# Autodesk Inventor assembly: Working Simlation and Assembly
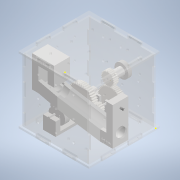
[picture p0: Inventor's stored thumbnail of the model, 180x180]
Saved by Autodesk Inventor 2021 (Build 250183000, 183)
## iProperties
Created: 2021-04-14
Part Number: Working Simlation and Assembly
Document SubType Name: Assembly
Designer: Nabeel Azafer
Author: Nabeel Azafer
## Documents named in this file (24)
- C:\Uni\Sem1\334\Project A\New Founding\ZIP\Working Simlation and Assembly.iam
- C:\Uni\Sem1\334\Project A\Spur Gear Large 4-1.ipt
- C:\Uni\Sem1\334\Project A\Spur Gear Small 4-1.ipt
- C:\Uni\Sem1\334\Project A\Block.ipt
- C:\Uni\Sem1\334\Project A\Cam.ipt
- C:\Uni\Sem1\334\Project A\Extra Shaft.ipt
- C:\Uni\Sem1\334\Project A\Shaft 2.ipt
- C:\Uni\Sem1\334\Project A\Spur Gear Small 2-1.ipt
- C:\Uni\Sem1\334\Project A\Spur Gear Large 2-1.ipt
- C:\Uni\Sem1\334\Project A\Input Connection.ipt
- C:\Uni\Sem1\334\Project A\Driveshaft coupling end.ipt
- C:\Uni\Sem1\334\Project A\Box base.ipt
- C:\Uni\Sem1\334\Project A\Box side 2.ipt
- C:\Uni\Sem1\334\Project A\Box side 4.ipt
- C:\Uni\Sem1\334\Project A\Box top.ipt
- C:\Uni\Sem1\334\Project A\Box side 1.ipt
- C:\Uni\Sem1\334\Project A\entry_ramp.ipt
- C:\Uni\Sem1\334\Project A\bottom_part.ipt
- C:\Uni\Sem1\334\Project A\Box_side_3.ipt
- C:\Uni\Sem1\334\Project A\Ball.ipt
- C:\Uni\Sem1\334\Project A\Support_1A.ipt
- C:\Uni\Sem1\334\Project A\Support_1B.ipt
- C:\Uni\Sem1\334\Project A\Support_2A.ipt
- C:\Uni\Sem1\334\Project A\Support_2B.ipt
## Components (23 placed, 21 different names)
1. Spur Gear1:1 — Mate:1, Flush:1, Rigid:1, Flush:4, Mate:2, Tangent:1, Rotation:1
2. Block:2 — Flush:2, Flush:3, Mate:24, Mate:25, Transitional:1
3. Cam:1 — Rigid:2, Flush:2, Transitional:1
4. Shaft 2:1 — Rigid:1, Rigid:2
5. Spur Gear2:1 — Flush:4, Mate:2, Tangent:1, Mate:3, Rotation:1, Rigid:3
6. Extra Shaft:2 — Rigid:3, Rigid:4
7. Spur Gear2:2 — Flush:7, Mate:4, Mate:5, Rigid:6, Rotation:2, Rigid:7, Mate:29
8. Spur Gear1:2 — Rigid:4, Flush:7, Mate:4, Rotation:2
9. Input Connection:1 — Rigid:5, Rigid:6, Rigid:7, Mate:28
10. Driveshaft coupling end:1 — Rigid:5
11. Box base:1 — Mate:9, Mate:10, Mate:11, Mate:13, Mate:14, Mate:27, Mate:28, Mate:31, Mate:32, Rigid:10, Rigid:12, Rigid:13
12. Box side 2:1 — Mate:12, Mate:13, Mate:14, Mate:15, Mate:23, Mate:30, Mate:33, Rigid:9
13. Box top:1 — Mate:22, Mate:23, Mate:30
14. Box side 1:1 — Mate:6, Mate:7, Mate:8, Mate:9, Mate:10, Mate:11, Mate:12, Mate:15, Rigid:11
15. Box side 4:2 — Mate:6, Mate:7, Mate:8, Mate:22, Rigid:8, Flush:10, Mate:29
16. entry_ramp:1 — Rigid:8, Mate:24, Mate:25
17. bottom_part:1 — Rigid:9
18. Box_side_3:1 — Mate:31, Mate:32, Mate:33
19. Ball:1
20. Support_1A:1 — Rigid:11
21. Support_1B:1 — Rigid:10, Flush:11
22. Support_2B:1 — Rigid:12
23. Support_2A:2 — Rigid:13
## Relationships (51: Mate 26, WeldJoint 13, Flush 8, RelateRotation 2, Tangent 1, Transitional 1)
- Mate:1: Spur Gear1:1
- Flush:1: Spur Gear1:1
- Rigid:1 [WeldJoint] (16 mm): Spur Gear1:1 ↔ Shaft 2:1
- Rigid:2 [WeldJoint] (-9.5 mm): Cam:1 ↔ Shaft 2:1
- Flush:2 (-4.5 mm): Block:2 ↔ Cam:1
- Flush:3 (-2.5 mm): Block:2
- Flush:4: Spur Gear1:1 ↔ Spur Gear2:1
- Mate:2: Spur Gear1:1 ↔ Spur Gear2:1
- Tangent:1: Spur Gear1:1 ↔ Spur Gear2:1
- Mate:3: Spur Gear2:1
- Rotation:1 [RelateRotation] (0.5 ul): Spur Gear1:1 ↔ Spur Gear2:1
- Rigid:3 [WeldJoint] (6.5 mm): Spur Gear2:1 ↔ Extra Shaft:2
- Rigid:4 [WeldJoint] (-6 mm): Extra Shaft:2 ↔ Spur Gear1:2
- Flush:6 (24.981 mm)
- Flush:7: Spur Gear2:2 ↔ Spur Gear1:2
- Mate:4: Spur Gear2:2 ↔ Spur Gear1:2
- Mate:5: Spur Gear2:2
- Rigid:5 [WeldJoint]: Input Connection:1 ↔ Driveshaft coupling end:1
- Rigid:6 [WeldJoint]: Spur Gear2:2 ↔ Input Connection:1
- Rotation:2 [RelateRotation] (0.5 ul): Spur Gear2:2 ↔ Spur Gear1:2
- Rigid:7 [WeldJoint]: Spur Gear2:2 ↔ Input Connection:1
- Mate:6: Box side 1:1 ↔ Box side 4:2
- Mate:7: Box side 1:1 ↔ Box side 4:2
- Mate:8: Box side 1:1 ↔ Box side 4:2
- Mate:9: Box base:1 ↔ Box side 1:1
- Mate:10: Box base:1 ↔ Box side 1:1
- Mate:11: Box base:1 ↔ Box side 1:1
- Mate:12: Box side 2:1 ↔ Box side 1:1
- Mate:13: Box base:1 ↔ Box side 2:1
- Mate:14: Box base:1 ↔ Box side 2:1
- Mate:15: Box side 2:1 ↔ Box side 1:1
- Mate:22: Box top:1 ↔ Box side 4:2
- Mate:23: Box side 2:1 ↔ Box top:1
- Rigid:8 [WeldJoint]: Box side 4:2 ↔ entry_ramp:1
- Mate:24 (0.5 mm): Block:2 ↔ entry_ramp:1
- Mate:25 (0.5 mm): Block:2 ↔ entry_ramp:1
- Flush:10 (48.343 mm): Box side 4:2
- Mate:27 (24 mm): Box base:1
- Mate:28 (48.516 mm): Input Connection:1 ↔ Box base:1
- Mate:29 (48.343 mm): Spur Gear2:2 ↔ Box side 4:2
- Mate:30: Box side 2:1 ↔ Box top:1
- Mate:31: Box base:1 ↔ Box_side_3:1
- Mate:32: Box base:1 ↔ Box_side_3:1
- Mate:33: Box side 2:1 ↔ Box_side_3:1
- Rigid:9 [WeldJoint]: Box side 2:1 ↔ bottom_part:1
- Rigid:10 [WeldJoint]: Box base:1 ↔ Support_1B:1
- Flush:11 (-2.962 mm): Support_1B:1
- Rigid:11 [WeldJoint]: Box side 1:1 ↔ Support_1A:1
- Rigid:12 [WeldJoint]: Box base:1 ↔ Support_2B:1
- Rigid:13 [WeldJoint]: Box base:1 ↔ Support_2A:2
- Transitional:1: Block:2 ↔ Cam:1
